# Autodesk Inventor assembly: robot_v2_turnigy
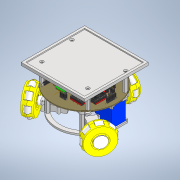
[picture p0: Inventor's stored thumbnail of the model, 180x180]
Saved by Autodesk Inventor 2020.2 (Build 242310000, 310)
## iProperties
Created: 2021-05-30
Part Number: robot_v2_turnigy
Document SubType Name: Assembly
Designer: Tarsoly
Author: Tarsoly
## Documents named in this file (10)
- D:\Users\Tarsoly\Dokumentumok\BME\Dipterv\3d\robot_v2_turnigy.iam
- D:\Users\Tarsoly\Dokumentumok\BME\Dipterv\3d\bottom2_turnigy.ipt
- D:\Users\Tarsoly\Dokumentumok\BME\Dipterv\3d\turnigy_battery.ipt
- D:\Users\Tarsoly\Dokumentumok\BME\Dipterv\3d\tavtarto_30mm.ipt
- D:\Users\Tarsoly\Dokumentumok\BME\Dipterv\3d\motor_top_v2.ipt
- D:\Users\Tarsoly\Dokumentumok\BME\Dipterv\3d\electronics.iam
- D:\Users\Tarsoly\Dokumentumok\BME\Dipterv\3d\top_v2.ipt
- D:\Users\Tarsoly\Dokumentumok\BME\Dipterv\3d\power_train_v2.iam
- D:\Users\Tarsoly\Dokumentumok\BME\Dipterv\3d\top_base.ipt
- D:\Users\Tarsoly\Dokumentumok\BME\Dipterv\3d\top_frame.ipt
## Components (21 placed, 9 different names)
1. bottom2_turnigy:1 — Mate:1, Mate:2, Angle:1, Mate:6, Mate:7, Mate:8, Mate:9, Mate:10, Mate:11, Mate:12, Mate:13, Mate:14, Mate:15, Mate:16, Mate:17, Mate:21, Mate:22, Mate:23, Mate:25, Mate:26, Mate:27, Mate:28, Mate:29, Mate:30, Mate:31, Mate:32, Mate:33
2. turnigy_battery:1 — Mate:6, Mate:7, Mate:8, Mate:18
3. tavtarto_30mm:1 — Mate:10, Mate:22
4. tavtarto_30mm:2 — Mate:11, Mate:21
5. tavtarto_30mm:3 — Mate:12, Mate:23
6. tavtarto_30mm:4 — Mate:9, Mate:16
7. electronics:1 [sub-assembly] — Angle:2, Mate:17, Mate:24
8. top_v2:1 — Mate:18, Mate:19, Mate:20, Mate:24
9. power_train_v2:1 [sub-assembly] — Mate:28, Mate:29, Mate:30
10. power_train_v2:2 [sub-assembly] — Mate:31, Mate:32, Mate:33
11. power_train_v2:3 [sub-assembly] — Mate:25, Mate:26, Mate:27
12. electronics:2 [sub-assembly] — Angle:3, Mate:39, Mate:40, Mate:41, Mate:42, Mate:43, Mate:44, Mate:45, Mate:46
13. tavtarto_30mm:5 — Mate:40, Mate:46
14. tavtarto_30mm:6 — Mate:41, Mate:45
15. tavtarto_30mm:7 — Mate:39, Mate:44, Mate:48, Mate:49
16. tavtarto_30mm:8 — Mate:42, Mate:43, Mate:47
17. top_base:1 — Mate:47, Mate:48, Mate:49, Mate:50
18. top_frame:1 — Flush:1, Flush:2, Mate:50
19. motor_top_v2:1 — Mate:13, Mate:14, Mate:15
20. motor_top_v2:2
21. motor_top_v2:3
## Component patterns: (3 elements, first: motor_top_v2:1)
## Relationships (47: Mate 42, Angle 3, Flush 2)
- Mate:1: bottom2_turnigy:1
- Mate:2: bottom2_turnigy:1
- Angle:1 (0 deg): bottom2_turnigy:1
- Mate:6: bottom2_turnigy:1 ↔ turnigy_battery:1
- Mate:7: bottom2_turnigy:1 ↔ turnigy_battery:1
- Mate:8: bottom2_turnigy:1 ↔ turnigy_battery:1
- Mate:9: bottom2_turnigy:1 ↔ tavtarto_30mm:4
- Mate:10: bottom2_turnigy:1 ↔ tavtarto_30mm:1
- Mate:11: bottom2_turnigy:1 ↔ tavtarto_30mm:2
- Mate:12: bottom2_turnigy:1 ↔ tavtarto_30mm:3
- Mate:13: bottom2_turnigy:1 ↔ motor_top_v2:1
- Mate:14: bottom2_turnigy:1 ↔ motor_top_v2:1
- Mate:15: bottom2_turnigy:1 ↔ motor_top_v2:1
- Mate:16: bottom2_turnigy:1 ↔ tavtarto_30mm:4
- Angle:2 (0 deg): electronics:1
- Mate:17: bottom2_turnigy:1 ↔ electronics:1
- Mate:18: turnigy_battery:1 ↔ top_v2:1
- Mate:19: top_v2:1
- Mate:20: top_v2:1
- Mate:21: bottom2_turnigy:1 ↔ tavtarto_30mm:2
- Mate:22: bottom2_turnigy:1 ↔ tavtarto_30mm:1
- Mate:23: bottom2_turnigy:1 ↔ tavtarto_30mm:3
- Mate:24: electronics:1 ↔ top_v2:1
- Mate:25: bottom2_turnigy:1 ↔ power_train_v2:3
- Mate:26: bottom2_turnigy:1 ↔ power_train_v2:3
- Mate:27: bottom2_turnigy:1 ↔ power_train_v2:3
- Mate:28: bottom2_turnigy:1 ↔ power_train_v2:1
- Mate:29: bottom2_turnigy:1 ↔ power_train_v2:1
- Mate:30: bottom2_turnigy:1 ↔ power_train_v2:1
- Mate:31: bottom2_turnigy:1 ↔ power_train_v2:2
- Mate:32: bottom2_turnigy:1 ↔ power_train_v2:2
- Mate:33: bottom2_turnigy:1 ↔ power_train_v2:2
- Angle:3 (0 deg): electronics:2
- Mate:39: electronics:2 ↔ tavtarto_30mm:7
- Mate:40: electronics:2 ↔ tavtarto_30mm:5
- Mate:41: electronics:2 ↔ tavtarto_30mm:6
- Mate:42: electronics:2 ↔ tavtarto_30mm:8
- Mate:43: electronics:2 ↔ tavtarto_30mm:8
- Mate:44: electronics:2 ↔ tavtarto_30mm:7
- Mate:45: electronics:2 ↔ tavtarto_30mm:6
- Mate:46: electronics:2 ↔ tavtarto_30mm:5
- Mate:47: tavtarto_30mm:8 ↔ top_base:1
- Mate:48: tavtarto_30mm:7 ↔ top_base:1
- Mate:49: tavtarto_30mm:7 ↔ top_base:1
- Flush:1: top_frame:1
- Flush:2: top_frame:1
- Mate:50: top_base:1 ↔ top_frame:1
